# Autodesk Inventor assembly: Sharp 2Y0A02 Assembled Case
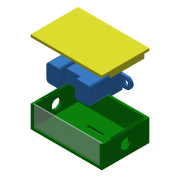
[picture p0: Inventor's stored thumbnail of the model, 180x180]
Saved by Autodesk Inventor 2018.3 (Build 223284000, 284)
## iProperties
Created: 2018-12-17
Part Number: Sharp 2Y0A02 Assembled Case
Document SubType Name: Assembly
Designer: aye06091
Mass: 15.5722 g
Surface Area: 155.118 cm^2
Volume: 14.9777 cm^3
Density: 1.03969 g/cm^3
Author: aye06091
## Documents named in this file (6)
- Y:\DeSimony-R\Senior R&D\4 R&D Shared Folder\VisiStick\VisiStick (Inventor)\Physical Parts\Sharp 2Y0A02 Assembled Case.iam
- Y:\DeSimony-R\Senior R&D\4 R&D Shared Folder\VisiStick\VisiStick (Inventor)\Physical Parts\Sharp 2Y0A02 Case.ipt
- Y:\DeSimony-R\Senior R&D\4 R&D Shared Folder\VisiStick\VisiStick (Inventor)\Physical Parts\Sharp 2Y0A02 Case Lid.ipt
- Y:\DeSimony-R\Senior R&D\4 R&D Shared Folder\VisiStick\VisiStick (Inventor)\Electronics\Sharp 2Y0A02.ipt
- Y:\DeSimony-R\Senior R&D\4 R&D Shared Folder\VisiStick\VisiStick (Inventor)\Physical Parts\Sharp 2Y0A02 Case Screen.ipt
- Y:\DeSimony-R\Senior R&D\4 R&D Shared Folder\VisiStick\VisiStick (Inventor)\Physical Parts\Sharp 2Y0A02 Case Weight.ipt
## Components (6 placed, 5 different names)
1. Sharp 2Y0A02 Case:1 — Flush:1, Mate:1, Mate:2, Mate:3, Mate:4, Mate:5, Mate:6, Mate:7, Mate:8, Flush:3
2. Sharp 2Y0A02 Case Lid:1 — Flush:1, Mate:1
3. Sharp 2Y0A02:1 — Mate:2, Mate:3
4. Sharp 2Y0A02 Case Screen:1 — Mate:4, Mate:5, Mate:6
5. Sharp 2Y0A02 Case Weight:1 — Mate:8, Mate:9, Flush:2
6. Sharp 2Y0A02 Case Weight:2 — Mate:7, Mate:9, Flush:2, Flush:3
## Relationships (12: Mate 9, Flush 3)
- Flush:1: Sharp 2Y0A02 Case:1 ↔ Sharp 2Y0A02 Case Lid:1
- Mate:1: Sharp 2Y0A02 Case:1 ↔ Sharp 2Y0A02 Case Lid:1
- Mate:2: Sharp 2Y0A02 Case:1 ↔ Sharp 2Y0A02:1
- Mate:3: Sharp 2Y0A02 Case:1 ↔ Sharp 2Y0A02:1
- Mate:4: Sharp 2Y0A02 Case:1 ↔ Sharp 2Y0A02 Case Screen:1
- Mate:5: Sharp 2Y0A02 Case:1 ↔ Sharp 2Y0A02 Case Screen:1
- Mate:6: Sharp 2Y0A02 Case:1 ↔ Sharp 2Y0A02 Case Screen:1
- Mate:7: Sharp 2Y0A02 Case:1 ↔ Sharp 2Y0A02 Case Weight:2
- Mate:8: Sharp 2Y0A02 Case:1 ↔ Sharp 2Y0A02 Case Weight:1
- Mate:9: Sharp 2Y0A02 Case Weight:1 ↔ Sharp 2Y0A02 Case Weight:2
- Flush:2: Sharp 2Y0A02 Case Weight:1 ↔ Sharp 2Y0A02 Case Weight:2
- Flush:3 (11.1379 mm): Sharp 2Y0A02 Case:1 ↔ Sharp 2Y0A02 Case Weight:2
